# Autodesk Inventor assembly: OpenVWheel
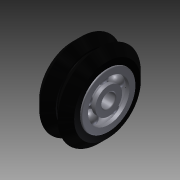
[picture p0: Inventor's stored thumbnail of the model, 180x180]
Saved by Autodesk Inventor 2014 (Build 180170000, 170)
## iProperties
Created: 2014-01-11
Part Number: OpenVWheel
Document SubType Name: Assembly
Designer: ThatOtherGuy
Mass: 12.5391 g
Surface Area: 39.9834 cm^2
Volume: 3.09274 cm^3
Density: 4.05438 g/cm^3
Author: ThatOtherGuy
## Documents named in this file (3)
- C:\Users\ThatOtherGuy\Documents\Inventor\KosselCNC1515\Carriage\OpenVWheel.iam
- C:\Users\ThatOtherGuy\Documents\Inventor\KosselCNC1515\Carriage\OpenVWheel.ipt
- C:\Users\ThatOtherGuy\Documents\Inventor\Content Center Files\R2014\en-US\DIN BEARING(1)\DIN 625 SKF - SKF 634.ipt
## Components (3 placed, 2 different names)
1. OpenVWheel:1 — Mate:1, Mate:2, Mate:3, Mate:4
2. DIN 625 SKF 634:3 — Mate:1, Mate:2
3. DIN 625 SKF 634:4 — Mate:3, Mate:4
## Relationships (4: Mate 4)
- Mate:2: OpenVWheel:1 ↔ DIN 625 SKF 634:3
- Mate:4: OpenVWheel:1 ↔ DIN 625 SKF 634:4
- Mate:1: OpenVWheel:1 ↔ DIN 625 SKF 634:3
- Mate:3: OpenVWheel:1 ↔ DIN 625 SKF 634:4
